# Autodesk Inventor assembly: mini sand
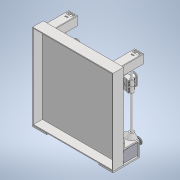
[picture p0: Inventor's stored thumbnail of the model, 180x180]
Saved by Autodesk Inventor 2022 (Build 260153000, 153)
## iProperties
Created: 2022-04-23
Part Number: mini sand
Document SubType Name: Assembly
Designer: Administrator
Title: mini sand v11
Author: Administrator
## Documents named in this file (17)
- Y:\Projects\Mini_Sand_Table\Mini Sand Table.iam
- Y:\Projects\Mini_Sand_Table\4mm x 140mm Rod.ipt
- Y:\Projects\Mini_Sand_Table\4mm x 8mm x 8mm Bushing.ipt
- Y:\Projects\Mini_Sand_Table\roller bearing.ipt
- Y:\Projects\Mini_Sand_Table\4mm x 130mm Rod.ipt
- Y:\Projects\Mini_Sand_Table\GT2 16T Pulley.ipt
- Y:\Projects\Mini_Sand_Table\Idle Bearing Mount.ipt
- Y:\Projects\Mini_Sand_Table\Magnet Mount.ipt
- Y:\Projects\Mini_Sand_Table\magnet.ipt
- Y:\Projects\Mini_Sand_Table\XY Joiner.ipt
- Y:\Projects\Mini_Sand_Table\LM4UU.ipt
- Y:\Projects\Mini_Sand_Table\Table Top.ipt
- Y:\Projects\Mini_Sand_Table\NEMA 11.ipt
- Y:\Projects\Mini_Sand_Table\Belt Retainer.ipt
- Y:\Projects\Mini_Sand_Table\Magnet Mount Lower.ipt
- Y:\Projects\Mini_Sand_Table\SKR PICO.ipt
- Y:\Projects\Mini_Sand_Table\Motor Mount.ipt
## Components (33 placed, 17 different names)
1. roller bearing:1 — Insert:11, Insert:50
2. roller bearing:2 — Insert:10, Insert:51
3. bushing:5 — Mate:13, Insert:43
4. bushing:6 — Mate:12, Insert:42
5. gt2 pulley 16t v1:1 — Insert:17
6. table mount (1):1 — Insert:16, Insert:24, Insert:25, Insert:31
7. roller bearing:3 — Insert:16
8. table mount (1):2 — Insert:23, Insert:26, Insert:27, Insert:30
9. roller bearing:4 — Insert:23
10. magnet:1 — Insert:44
11. magnet mount:1 — Insert:42, Insert:43, Insert:44, Insert:45, Insert:46
12. XY Joiner:1 — Insert:3, Insert:4, Insert:10, Insert:11, Mate:11
13. LM4UU:1 — Insert:3
14. LM4UU:2 — Insert:4, Mate:10
15. LM4UU:3 — Insert:5, Mate:9
16. LM4UU:4 — Insert:6
17. XY Joiner:2 — Insert:5, Insert:6, Insert:34, Insert:35, Insert:40, Insert:41
18. 4mm x 140mm Rod:1 — Insert:31, Mate:10, Mate:18
19. 4mm x 140mm Rod:2 — Mate:9, Insert:30, Mate:19
20. Table Top:1 — Insert:24, Insert:25, Insert:26, Insert:27, Mate:14, Mate:15, Mate:20, Mate:21, Mate:22
21. NEMA 11:1 — Insert:29, Insert:48, Insert:49
22. NEMA 11:2 — Insert:17, Mate:17, Insert:47
23. GT2 16T Pulley:2 — Insert:29
24. 4mm x 130mm Rod:2 — Insert:40, Mate:11, Mate:13
25. Belt Retainer:1 — Insert:52, Insert:53
26. Belt Retainer:2 — Insert:50, Insert:51
27. roller bearing:5 — Insert:35, Insert:52
28. roller bearing:6 — Insert:34, Insert:53
29. Magnet Mount Lower:1 — Insert:45, Insert:46
30. 4mm x 130mm Rod:3 — Insert:41, Mate:12
31. SKR PICO:1 — Mate:14
32. Motor Mount:1 — Mate:15, Mate:17, Insert:47, Mate:18, Mate:21
33. Motor Mount:2 — Insert:48, Insert:49, Mate:19, Mate:20, Mate:22
## Relationships (45: Insert 32, Mate 13)
- Insert:3: XY Joiner:1 ↔ LM4UU:1
- Insert:4: XY Joiner:1 ↔ LM4UU:2
- Insert:5: LM4UU:3 ↔ XY Joiner:2
- Insert:6: LM4UU:4 ↔ XY Joiner:2
- Insert:10: roller bearing:2 ↔ XY Joiner:1
- Insert:11: roller bearing:1 ↔ XY Joiner:1
- Insert:16: table mount (1):1 ↔ roller bearing:3
- Insert:17: gt2 pulley 16t v1:1 ↔ NEMA 11:2
- Insert:23: table mount (1):2 ↔ roller bearing:4
- Insert:24: table mount (1):1 ↔ Table Top:1
- Insert:25: table mount (1):1 ↔ Table Top:1
- Insert:26: table mount (1):2 ↔ Table Top:1
- Insert:27: table mount (1):2 ↔ Table Top:1
- Insert:29: NEMA 11:1 ↔ GT2 16T Pulley:2
- Mate:9: LM4UU:3 ↔ 4mm x 140mm Rod:2
- Insert:30: table mount (1):2 ↔ 4mm x 140mm Rod:2
- Insert:31: table mount (1):1 ↔ 4mm x 140mm Rod:1
- Mate:10: LM4UU:2 ↔ 4mm x 140mm Rod:1
- Insert:34: XY Joiner:2 ↔ roller bearing:6
- Insert:35: XY Joiner:2 ↔ roller bearing:5
- Insert:40: XY Joiner:2 ↔ 4mm x 130mm Rod:2
- Insert:41: XY Joiner:2 ↔ 4mm x 130mm Rod:3
- Mate:11: XY Joiner:1 ↔ 4mm x 130mm Rod:2
- Mate:12: bushing:6 ↔ 4mm x 130mm Rod:3
- Mate:13: bushing:5 ↔ 4mm x 130mm Rod:2
- Insert:42 (-2 mm): bushing:6 ↔ magnet mount:1
- Insert:43 (2 mm): bushing:5 ↔ magnet mount:1
- Insert:44: magnet:1 ↔ magnet mount:1
- Insert:45: magnet mount:1 ↔ Magnet Mount Lower:1
- Insert:46: magnet mount:1 ↔ Magnet Mount Lower:1
- Mate:14: Table Top:1 ↔ SKR PICO:1
- Mate:15: Table Top:1 ↔ Motor Mount:1
- Mate:17: NEMA 11:2 ↔ Motor Mount:1
- Insert:47: NEMA 11:2 ↔ Motor Mount:1
- Insert:48: NEMA 11:1 ↔ Motor Mount:2
- Insert:49: NEMA 11:1 ↔ Motor Mount:2
- Mate:18: 4mm x 140mm Rod:1 ↔ Motor Mount:1
- Mate:19: 4mm x 140mm Rod:2 ↔ Motor Mount:2
- Mate:20: Table Top:1 ↔ Motor Mount:2
- Mate:21: Table Top:1 ↔ Motor Mount:1
- Insert:50: roller bearing:1 ↔ Belt Retainer:2
- Insert:51: roller bearing:2 ↔ Belt Retainer:2
- Insert:52: Belt Retainer:1 ↔ roller bearing:5
- Insert:53: Belt Retainer:1 ↔ roller bearing:6
- Mate:22: Table Top:1 ↔ Motor Mount:2
